# Autodesk Inventor assembly: ASSEMBLY_Bottom_Cone_Rod
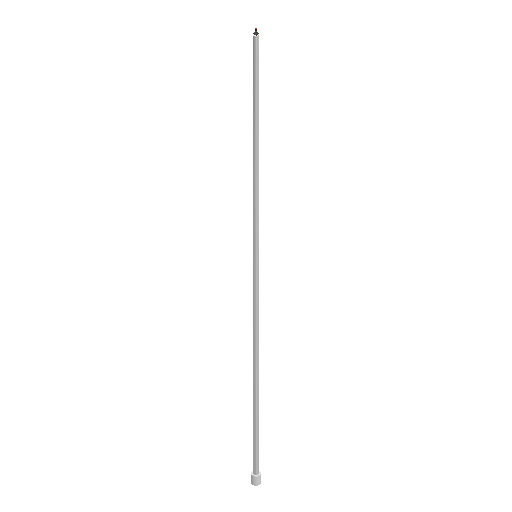
[picture p0: Inventor's stored thumbnail of the model, 512x512]
Saved by Autodesk Inventor 2026.1 (Build 301233000, 233)
## iProperties
Created: 2025-06-19
Part Number: ASSEMBLY_Bottom_Cone_Rod
Document SubType Name: Assembly
Designer: User
Author: User
## Documents named in this file (5)
- C:\Users\Andrzej\OneDrive\_DRIVE_SYNCH_FILES\__ BYTECHLAB PROJECTS\RF - Mostly 3D Printed Discone Antenna\MCAD\15_DISCONE_V4\ASSEMBLY_MAIN_REVA\ASSEMBLY_Bottom_Cone_Rod.iam
- C:\Users\Andrzej\OneDrive\_DRIVE_SYNCH_FILES\__ BYTECHLAB PROJECTS\RF - Mostly 3D Printed Discone Antenna\MCAD\15_DISCONE_V4\__CONTENT_CENTER_PARTS\en-US\ISO 7380-1\ISO 7380-1 - M4 x 10.ipt
- C:\Users\Andrzej\OneDrive\_DRIVE_SYNCH_FILES\__ BYTECHLAB PROJECTS\RF - Mostly 3D Printed Discone Antenna\MCAD\15_DISCONE_V4\ASSEMBLY_MAIN_REVA\CUT_ALU_10x800mm_Rod.ipt
- C:\Users\Andrzej\OneDrive\_DRIVE_SYNCH_FILES\__ BYTECHLAB PROJECTS\RF - Mostly 3D Printed Discone Antenna\MCAD\15_DISCONE_V4\ASSEMBLY_MAIN_REVA\CUT_COPPER_Bottom_Cone_1,5mm_Connecting_Wire.ipt
- C:\Users\Andrzej\OneDrive\_DRIVE_SYNCH_FILES\__ BYTECHLAB PROJECTS\RF - Mostly 3D Printed Discone Antenna\MCAD\15_DISCONE_V4\ASSEMBLY_MAIN_REVA\3DP_ASA_Rod_End_Cap.ipt
## Components (4 placed, 4 different names)
1. CUT_ALU_10x800mm_Rod:1 — Mate:1, Mate:2, Mate:3, Mate:5, Mate:6
2. CUT_COPPER_Bottom_Cone_1,5mm_Connecting_Wire:1 — Mate:2, Mate:4
3. ISO 7380-1 M4 x 10:1 — Mate:3, Mate:4, Mate:1
4. 3DP_ASA_Rod_End_Cap:1 — Mate:5, Mate:6
## Relationships (6: Mate 6)
- Mate:1: CUT_ALU_10x800mm_Rod:1 ↔ ISO 7380-1 M4 x 10:1
- Mate:2: CUT_ALU_10x800mm_Rod:1 ↔ CUT_COPPER_Bottom_Cone_1,5mm_Connecting_Wire:1
- Mate:3: CUT_ALU_10x800mm_Rod:1 ↔ ISO 7380-1 M4 x 10:1
- Mate:4: CUT_COPPER_Bottom_Cone_1,5mm_Connecting_Wire:1 ↔ ISO 7380-1 M4 x 10:1
- Mate:5: CUT_ALU_10x800mm_Rod:1 ↔ 3DP_ASA_Rod_End_Cap:1
- Mate:6: CUT_ALU_10x800mm_Rod:1 ↔ 3DP_ASA_Rod_End_Cap:1
